# Autodesk Inventor assembly: Assembly
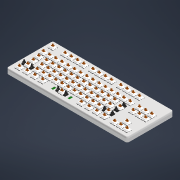
[picture p0: Inventor's stored thumbnail of the model, 180x180]
Saved by Autodesk Inventor 2022 (Build 260153000, 153)
## iProperties
Created: 2021-09-25
Part Number: Assembly
Document SubType Name: Weldment
Designer: shiok
Weld Material: Welded Aluminum-6061
Author: shiok
## Documents named in this file (4)
- C:\Users\shiok\Documents\GitHub\Keyboard_H\chassis\2022\Assembly.iam
- C:\Users\shiok\Documents\GitHub\Keyboard_H\chassis\2022\Base.ipt
- C:\Users\shiok\Documents\GitHub\Keyboard_H\chassis\2022\Plate.ipt
- C:\Users\shiok\Documents\GitHub\Keyboard_H\pcb\3D_model\step\keyboard_h.iam
## Components (3 placed, 3 different names)
1. Plate:1 — メイト:1, メイト:2, メイト:3, フラッシュ:1, フラッシュ:2
2. keyboard_h:1 [sub-assembly] — メイト:1, メイト:2, メイト:3, メイト:4
3. Base:1 — フラッシュ:1, フラッシュ:2, メイト:4
## Relationships (6: Mate 4, Flush 2)
- メイト:1 [Mate]: Plate:1 ↔ keyboard_h:1
- メイト:2 [Mate]: Plate:1 ↔ keyboard_h:1
- メイト:3 [Mate]: Plate:1 ↔ keyboard_h:1
- フラッシュ:1 [Flush]: Plate:1 ↔ Base:1
- フラッシュ:2 [Flush]: Plate:1 ↔ Base:1
- メイト:4 [Mate]: keyboard_h:1 ↔ Base:1
